# Autodesk Inventor assembly: RightUpperLimbBlock
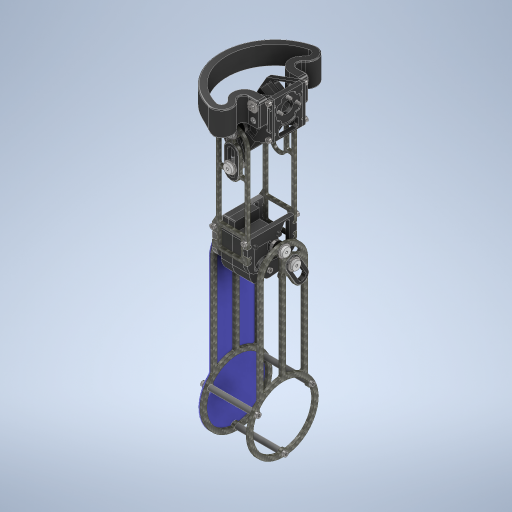
[picture p0: Inventor's stored thumbnail of the model, 512x512]
Saved by Autodesk Inventor 2024.2 (Build 282272000, 272)
## iProperties
Created: 2024-01-18
Part Number: RightUpperLimbBlock
Document SubType Name: Assembly
Designer: Masato Kubotera
Mass: 424.438 g
Surface Area: 1330.22 cm^2
Volume: 215.834 cm^3
Density: 1.9665 g/cm^3
Author: Masato Kubotera
## Documents named in this file (6)
- C:\Users\masato\OneDrive - Chiba Institute of Technology\CIT Brains\RoboCup2024\SUSTAINA-OP2-DEV\NativeFiles\Boby\UpperLimb\RightUpperLimbBlock.iam
- C:\Users\masato\OneDrive - Chiba Institute of Technology\CIT Brains\RoboCup2024\SUSTAINA-OP2-DEV\NativeFiles\Boby\UpperLimb\Shoulders\RightShoulderUnit.iam
- C:\Users\masato\OneDrive - Chiba Institute of Technology\CIT Brains\RoboCup2024\SUSTAINA-OP2-DEV\NativeFiles\Boby\UpperLimb\UpperArms\RightUpperArmUnit.iam
- C:\Users\masato\OneDrive - Chiba Institute of Technology\CIT Brains\RoboCup2024\SUSTAINA-OP2-DEV\NativeFiles\Boby\UpperLimb\Shoulders\RightShoulderCrankUnit.iam
- C:\Users\masato\OneDrive - Chiba Institute of Technology\CIT Brains\RoboCup2024\SUSTAINA-OP2-DEV\NativeFiles\Boby\UpperLimb\LowerArms\RightLowerArmUnit.iam
- C:\Users\masato\OneDrive - Chiba Institute of Technology\CIT Brains\RoboCup2024\SUSTAINA-OP2-DEV\NativeFiles\Boby\UpperLimb\UpperArms\RightUpperArmCrankUnit.iam
## Components (5 placed, 5 different names)
1. RightShoulderUnit:1 [sub-assembly] — Shoulder-Pitch, Shoulder-Roll, [Auto]Shoulder-Roll-Crank, Mate:1, Flush:1, Insert:1, Insert:2, Insert:3
2. RightShoulderCrankUnit:1 [sub-assembly] — Insert:1, [Auto]Shoulder-Roll-Crank
3. RightUpperArmUnit:1 [sub-assembly] — Insert:2, Insert:3, Shoulder-Roll, Elbow-Pitch, Insert:4, Insert:5, [Auto]Elbow-Pitch, Insert:6
4. RightUpperArmCrankUnit:1 [sub-assembly] — Insert:5, [Auto]Elbow-Pitch
5. RightLowerArmUnit:1 [sub-assembly] — Insert:4, Insert:6, Elbow-Pitch
## Relationships (13: Insert 6, Angle 5, Mate 1, Flush 1)
- Shoulder-Pitch [Angle] (0 deg): RightShoulderUnit:1
- Shoulder-Roll [Angle] (0 deg): RightShoulderUnit:1 ↔ RightUpperArmUnit:1
- Elbow-Pitch [Angle] (0 deg): RightUpperArmUnit:1 ↔ RightLowerArmUnit:1
- [Auto]Shoulder-Roll-Crank [Angle] (180 deg): RightShoulderUnit:1 ↔ RightShoulderCrankUnit:1
- [Auto]Elbow-Pitch [Angle] (-180 deg): RightUpperArmUnit:1 ↔ RightUpperArmCrankUnit:1
- Insert:6: RightUpperArmUnit:1 ↔ RightLowerArmUnit:1
- Mate:1: RightShoulderUnit:1
- Flush:1: RightShoulderUnit:1
- Insert:1: RightShoulderUnit:1 ↔ RightShoulderCrankUnit:1
- Insert:2: RightShoulderUnit:1 ↔ RightUpperArmUnit:1
- Insert:3: RightShoulderUnit:1 ↔ RightUpperArmUnit:1
- Insert:4: RightUpperArmUnit:1 ↔ RightLowerArmUnit:1
- Insert:5: RightUpperArmUnit:1 ↔ RightUpperArmCrankUnit:1
